# Autodesk Inventor assembly: ASSY,INTAKE,LINEAR
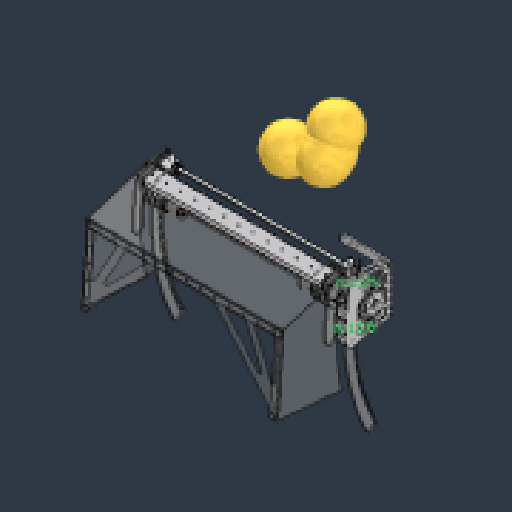
[picture p0: Inventor's stored thumbnail of the model, 512x512]
Saved by Autodesk Inventor 2026 (Build 300175050, 175E)
## iProperties
Created: 2026-04-11
Part Number: ASSY,INTAKE,LINEAR
Document SubType Name: Assembly
Designer: Jthib
Mass: 12352.9 g
Surface Area: 19154.1 cm^2
Volume: 9875.56 cm^3
Density: 1.25086 g/cm^3
Author: Jthib
## Documents named in this file (27)
- C:\Users\Jthib\Documents\GitHub\2026-Robot-Mechanical\LINEAR_INTAKE\ASSY,INTAKE,LINEAR.iam
- C:\Users\Jthib\Documents\GitHub\2026-Robot-Mechanical\#2_2026 Field CAD\GE-26900_ Fuel.ipt
- C:\Users\Jthib\Documents\GitHub\2026-Robot-Mechanical\Intake\PLATE,CLAMP,MK4i,Swerve,CUSTOM,FRC2026.ipt
- C:\Users\Jthib\Documents\GitHub\2026-Robot-Mechanical\LINEAR_INTAKE\PLATE,SIDE,INTAKE,FRONT.ipt
- C:\Users\Jthib\Documents\GitHub\2026-Robot-Mechanical\LINEAR_INTAKE\#old-linear-intake\INSIDE_INTAKE_PLATE.ipt
- C:\Users\Jthib\Documents\GitHub\2026-Robot-Mechanical\LINEAR_INTAKE\#old-linear-intake\FRONT_INTAKE_LEXAN.ipt
- C:\Users\Jthib\Documents\GitHub\2026-Robot-Mechanical\LINEAR_INTAKE\#old-linear-intake\SIDE_INTAKE_LEXAN.ipt
- C:\Users\Jthib\Documents\GitHub\2026-Robot-Mechanical\LINEAR_INTAKE\#old-linear-intake\SIDE_INTAKE_LEXAN_MIR.ipt
- C:\Users\Jthib\Documents\GitHub\2026-Robot-Mechanical\LINEAR_INTAKE\#old-linear-intake\TOP_INTAKE_LEXAN.ipt
- C:\Users\Jthib\Documents\GitHub\2026-Robot-Mechanical\#1_CAD Library\Power Transmission\Bearings\PURCHASED,HEX_BEARING.ipt
- C:\Users\Jthib\Documents\GitHub\2026-Robot-Mechanical\LINEAR_INTAKE\#old-linear-intake\INTAKE_DRIVEN_PULLY.ipt
- C:\Users\Jthib\Documents\GitHub\2026-Robot-Mechanical\LINEAR_INTAKE\#old-linear-intake\INSIDE_INTAKE_PLATE_MOTOR_MOUNT.ipt
- C:\Users\Jthib\Documents\GitHub\2026-Robot-Mechanical\LINEAR_INTAKE\#old-linear-intake\INSIDE_INTAKE_PLATE_MOTOR_MOUNT_MIR.ipt
- C:\Users\Jthib\Documents\GitHub\2026-Robot-Mechanical\LINEAR_INTAKE\#old-linear-intake\53t_Belt.ipt
- C:\Users\Jthib\Documents\GitHub\2026-Robot-Mechanical\LINEAR_INTAKE\#old-linear-intake\MOTOR_PLATE_PRINTED_SPACER.ipt
- C:\Users\Jthib\Documents\GitHub\2026-Robot-Mechanical\LINEAR_INTAKE\#old-linear-intake\OUTSIDE_INTAKE_SPACERS.ipt
- C:\Users\Jthib\Documents\GitHub\2026-Robot-Mechanical\LINEAR_INTAKE\#old-linear-intake\CRASH_BAR_INTAKE.ipt
- C:\Users\Jthib\Documents\GitHub\2026-Robot-Mechanical\#1_CAD Library\Electronics\CONTROLS,SPARK_FLEX.ipt
- C:\Users\Jthib\Documents\GitHub\2026-Robot-Mechanical\#1_CAD Library\Motors\MOTOR,REV,NEO,VORTEX.ipt
- C:\Users\Jthib\Documents\GitHub\2026-Robot-Mechanical\LINEAR_INTAKE\#old-linear-intake\INTAKE_DRIVER_PULLY.ipt
- C:\Users\Jthib\Documents\GitHub\2026-Robot-Mechanical\LINEAR_INTAKE\GEAR,PINION,INTAKE.ipt
- C:\Users\Jthib\Documents\GitHub\2026-Robot-Mechanical\Intake\STOCK,HEX,INTAKE.ipt
- C:\Users\Jthib\Documents\GitHub\2026-Robot-Mechanical\LINEAR_INTAKE\GEAR,DRIVE,INTAKE.ipt
- C:\Users\Jthib\Documents\GitHub\2026-Robot-Mechanical\LINEAR_INTAKE\SPACER,INTAKE,LINEAR.ipt
- C:\Users\Jthib\Documents\GitHub\2026-Robot-Mechanical\LINEAR_INTAKE\RACK,OUTSIDE.ipt
- C:\Users\Jthib\Documents\GitHub\2026-Robot-Mechanical\LINEAR_INTAKE\RACK,INSIDE.ipt
- C:\Users\Jthib\Documents\GitHub\2026-Robot-Mechanical\LINEAR_INTAKE\FRONT,HEX,INTAKE.ipt
## Components (42 placed, 26 different names)
1. PLATE,CLAMP,MK4i,Swerve,CUSTOM,FRC2026:1 — Mate:1, Mate:2, Mate:3, Mate:4, Mate:5
2. GE-26900_ Fuel:8
3. PLATE,SIDE,INTAKE,FRONT:1 — Mate:1, Mate:2, Mate:3, Flush:1, Mate:78, Mate:80, Mate:81, Mate:82, Mate:87, Mate:88, Mate:93
4. PLATE,SIDE,INTAKE,FRONT:2 — Mate:4, Flush:1, Mate:5, Mate:76, Insert:15
5. RACK,OUTSIDE:1 — Mate:76, Rotation:1, Rotation:2, Mate:89, Mate:90, Mate:91, Mate:93, Mate:99, Mate:100, Mate:101
6. INSIDE_INTAKE_PLATE:1 — Mate:38, Mate:41, Mate:42, Mate:49, Flush:21
7. INSIDE_INTAKE_PLATE:2 — Mate:31, Mate:47, Mate:49, Mate:79, Mate:92, Mate:105
8. FRONT_INTAKE_LEXAN:1 — Mate:73, Insert:7, Insert:8, Insert:9, Insert:10, Mate:97, Mate:98
9. SIDE_INTAKE_LEXAN:1 — Flush:20, Mate:97
10. SIDE_INTAKE_LEXAN_MIR:1 — Mate:98
11. TOP_INTAKE_LEXAN:1
12. PURCHASED,HEX_BEARING:1 — Mate:48, Mate:50, Mate:51
13. PURCHASED,HEX_BEARING:2 — Mate:48
14. INTAKE_DRIVEN_PULLY:1 — Mate:45
15. INSIDE_INTAKE_PLATE_MOTOR_MOUNT:1 — Mate:32, Mate:33, Mate:34, Mate:59, Mate:60, Mate:61, Insert:5, Insert:6
16. INSIDE_INTAKE_PLATE_MOTOR_MOUNT_MIR:1 — Mate:43, Mate:44, Insert:1, Insert:2, Mate:67, Insert:3, Insert:4
17. 53t_Belt:1 — Mate:45, Mate:68, Mate:69
18. 53t_Belt:2 — Mate:52, Mate:53, Mate:70, Mate:71
19. MOTOR_PLATE_PRINTED_SPACER:1 — Mate:38, Mate:41, Mate:42, Mate:43, Mate:44
20. MOTOR_PLATE_PRINTED_SPACER:2 — Mate:32, Mate:33, Mate:34, Mate:47
21. SPACER,INTAKE,LINEAR:1 — Mate:31, Mate:62, Mate:92, Mate:100, Mate:101, Mate:102
22. OUTSIDE_INTAKE_SPACERS:2
23. INTAKE_DRIVEN_PULLY:2 — Mate:50, Mate:51, Mate:52, Mate:53
24. CRASH_BAR_INTAKE:1 — Insert:3, Insert:4, Insert:5, Insert:6, Mate:73, Insert:7, Insert:8, Insert:9, Insert:10
25. CONTROLS,SPARK_FLEX:1 — Mate:59, Mate:60, Mate:61
26. MOTOR,REV,NEO,VORTEX:1
27. INTAKE_DRIVER_PULLY:1 — Mate:62, Mate:70, Mate:71
28. CONTROLS,SPARK_FLEX:2 — Insert:1, Insert:2
29. MOTOR,REV,NEO,VORTEX:2
30. INTAKE_DRIVER_PULLY:2 — Mate:67, Mate:68, Mate:69
31. PINION:1 — Mate:78, Rotation:1, Mate:82
32. STOCK,HEX,INTAKE:1 — Mate:79, Flush:20
33. PINION:2 — Mate:80, Mate:81, Rotation:2, Rotation:3
34. PURCHASED,HEX_BEARING:3 — Insert:15
35. GEAR,DRIVE,INTAKE:1 — Mate:87, Mate:88, Rotation:3
36. RACK,INSIDE:1 — Mate:89, Mate:90, Mate:91, Mate:99, Mate:102, Mate:103, Mate:104
37. RACK,OUTSIDE:2 — Mate:94, Mate:95, Mate:96
38. RACK,INSIDE:2 — Mate:94, Mate:95, Mate:96, Mate:103, Mate:104
39. GE-26900_ Fuel:9
40. GE-26900_ Fuel:10
41. GE-26900_ Fuel:11
42. FRONT,HEX,INTAKE:1 — Mate:105, Flush:21
## Relationships (103: Mate 76, Flush 13, Insert 11, RelateRotation 3)
- Mate:1: PLATE,CLAMP,MK4i,Swerve,CUSTOM,FRC2026:1 ↔ PLATE,SIDE,INTAKE,FRONT:1
- Mate:2 (0.127 mm): PLATE,CLAMP,MK4i,Swerve,CUSTOM,FRC2026:1 ↔ PLATE,SIDE,INTAKE,FRONT:1
- Mate:3 (0.1778 mm): PLATE,CLAMP,MK4i,Swerve,CUSTOM,FRC2026:1 ↔ PLATE,SIDE,INTAKE,FRONT:1
- Mate:4 (0.127 mm): PLATE,CLAMP,MK4i,Swerve,CUSTOM,FRC2026:1 ↔ PLATE,SIDE,INTAKE,FRONT:2
- Flush:1: PLATE,SIDE,INTAKE,FRONT:1 ↔ PLATE,SIDE,INTAKE,FRONT:2
- Mate:5: PLATE,CLAMP,MK4i,Swerve,CUSTOM,FRC2026:1 ↔ PLATE,SIDE,INTAKE,FRONT:2
- [Mate]: FRONT_INTAKE_LEXAN:1 ↔ SIDE_INTAKE_LEXAN:1
- [Flush]: FRONT_INTAKE_LEXAN:1 ↔ SIDE_INTAKE_LEXAN:1
- [Mate]: FRONT_INTAKE_LEXAN:1 ↔ SIDE_INTAKE_LEXAN_MIR:1
- [Flush]: FRONT_INTAKE_LEXAN:1 ↔ SIDE_INTAKE_LEXAN_MIR:1
- [Mate]: SIDE_INTAKE_LEXAN_MIR:1 ↔ TOP_INTAKE_LEXAN:1
- [Flush]: SIDE_INTAKE_LEXAN_MIR:1 ↔ TOP_INTAKE_LEXAN:1
- [Flush]: FRONT_INTAKE_LEXAN:1 ↔ TOP_INTAKE_LEXAN:1
- [Mate]: INSIDE_INTAKE_PLATE:2 ↔ PURCHASED,HEX_BEARING:1
- [Mate]: INSIDE_INTAKE_PLATE:2 ↔ PURCHASED,HEX_BEARING:1
- [Mate]: INSIDE_INTAKE_PLATE:1 ↔ PURCHASED,HEX_BEARING:2
- [Mate]: INSIDE_INTAKE_PLATE:1 ↔ PURCHASED,HEX_BEARING:2
- [Mate] (0.7937 mm): PURCHASED,HEX_BEARING:2 ↔ INTAKE_DRIVEN_PULLY:1
- [Mate]: PURCHASED,HEX_BEARING:2 ↔ INTAKE_DRIVEN_PULLY:1
- [Mate]: INTAKE_DRIVEN_PULLY:1 ↔ 53t_Belt:1
- [Mate]: INSIDE_INTAKE_PLATE_MOTOR_MOUNT_MIR:1 ↔ MOTOR_PLATE_PRINTED_SPACER:1
- [Mate]: INSIDE_INTAKE_PLATE:2 ↔ MOTOR_PLATE_PRINTED_SPACER:2
- [Flush]: INSIDE_INTAKE_PLATE:2 ↔ MOTOR_PLATE_PRINTED_SPACER:2
- [Flush]: INSIDE_INTAKE_PLATE_MOTOR_MOUNT_MIR:1 ↔ MOTOR_PLATE_PRINTED_SPACER:1
- [Flush]: INSIDE_INTAKE_PLATE:2 ↔ SPACER,INTAKE,LINEAR:1
- [Flush]: MOTOR_PLATE_PRINTED_SPACER:2 ↔ SPACER,INTAKE,LINEAR:1
- [Mate]: INSIDE_INTAKE_PLATE:1 ↔ OUTSIDE_INTAKE_SPACERS:2
- [Flush]: INSIDE_INTAKE_PLATE:1 ↔ OUTSIDE_INTAKE_SPACERS:2
- [Flush]: MOTOR_PLATE_PRINTED_SPACER:1 ↔ OUTSIDE_INTAKE_SPACERS:2
- Mate:31: INSIDE_INTAKE_PLATE:2 ↔ SPACER,INTAKE,LINEAR:1
- Mate:32: INSIDE_INTAKE_PLATE_MOTOR_MOUNT:1 ↔ MOTOR_PLATE_PRINTED_SPACER:2
- Mate:33: INSIDE_INTAKE_PLATE_MOTOR_MOUNT:1 ↔ MOTOR_PLATE_PRINTED_SPACER:2
- Mate:34: INSIDE_INTAKE_PLATE_MOTOR_MOUNT:1 ↔ MOTOR_PLATE_PRINTED_SPACER:2
- Mate:38: INSIDE_INTAKE_PLATE:1 ↔ MOTOR_PLATE_PRINTED_SPACER:1
- Mate:41: INSIDE_INTAKE_PLATE:1 ↔ MOTOR_PLATE_PRINTED_SPACER:1
- Mate:42: INSIDE_INTAKE_PLATE:1 ↔ MOTOR_PLATE_PRINTED_SPACER:1
- Mate:43: INSIDE_INTAKE_PLATE_MOTOR_MOUNT_MIR:1 ↔ MOTOR_PLATE_PRINTED_SPACER:1
- Mate:44: INSIDE_INTAKE_PLATE_MOTOR_MOUNT_MIR:1 ↔ MOTOR_PLATE_PRINTED_SPACER:1
- Mate:45: INTAKE_DRIVEN_PULLY:1 ↔ 53t_Belt:1
- Mate:47: INSIDE_INTAKE_PLATE:2 ↔ MOTOR_PLATE_PRINTED_SPACER:2
- Mate:48: PURCHASED,HEX_BEARING:1 ↔ PURCHASED,HEX_BEARING:2
- Mate:49: INSIDE_INTAKE_PLATE:1 ↔ INSIDE_INTAKE_PLATE:2
- Mate:50: PURCHASED,HEX_BEARING:1 ↔ INTAKE_DRIVEN_PULLY:2
- Mate:51: PURCHASED,HEX_BEARING:1 ↔ INTAKE_DRIVEN_PULLY:2
- Mate:52: 53t_Belt:2 ↔ INTAKE_DRIVEN_PULLY:2
- Mate:53: 53t_Belt:2 ↔ INTAKE_DRIVEN_PULLY:2
- [Mate]: CONTROLS,SPARK_FLEX:1 ↔ MOTOR,REV,NEO,VORTEX:1
- [Mate]: CONTROLS,SPARK_FLEX:1 ↔ MOTOR,REV,NEO,VORTEX:1
- [Mate]: CONTROLS,SPARK_FLEX:1 ↔ MOTOR,REV,NEO,VORTEX:1
- Mate:59: INSIDE_INTAKE_PLATE_MOTOR_MOUNT:1 ↔ CONTROLS,SPARK_FLEX:1
- Mate:60: INSIDE_INTAKE_PLATE_MOTOR_MOUNT:1 ↔ CONTROLS,SPARK_FLEX:1
- Mate:61: INSIDE_INTAKE_PLATE_MOTOR_MOUNT:1 ↔ CONTROLS,SPARK_FLEX:1
- Mate:62: SPACER,INTAKE,LINEAR:1 ↔ INTAKE_DRIVER_PULLY:1
- [Mate]: CONTROLS,SPARK_FLEX:2 ↔ MOTOR,REV,NEO,VORTEX:2
- [Mate]: CONTROLS,SPARK_FLEX:2 ↔ MOTOR,REV,NEO,VORTEX:2
- [Mate]: CONTROLS,SPARK_FLEX:2 ↔ MOTOR,REV,NEO,VORTEX:2
- Insert:1: INSIDE_INTAKE_PLATE_MOTOR_MOUNT_MIR:1 ↔ CONTROLS,SPARK_FLEX:2
- Insert:2: INSIDE_INTAKE_PLATE_MOTOR_MOUNT_MIR:1 ↔ CONTROLS,SPARK_FLEX:2
- Mate:67: INSIDE_INTAKE_PLATE_MOTOR_MOUNT_MIR:1 ↔ INTAKE_DRIVER_PULLY:2
- Mate:68: 53t_Belt:1 ↔ INTAKE_DRIVER_PULLY:2
- Mate:69: 53t_Belt:1 ↔ INTAKE_DRIVER_PULLY:2
- Mate:70: 53t_Belt:2 ↔ INTAKE_DRIVER_PULLY:1
- Mate:71: 53t_Belt:2 ↔ INTAKE_DRIVER_PULLY:1
- Insert:3: INSIDE_INTAKE_PLATE_MOTOR_MOUNT_MIR:1 ↔ CRASH_BAR_INTAKE:1
- Insert:4: INSIDE_INTAKE_PLATE_MOTOR_MOUNT_MIR:1 ↔ CRASH_BAR_INTAKE:1
- Insert:5: INSIDE_INTAKE_PLATE_MOTOR_MOUNT:1 ↔ CRASH_BAR_INTAKE:1
- Insert:6: INSIDE_INTAKE_PLATE_MOTOR_MOUNT:1 ↔ CRASH_BAR_INTAKE:1
- Mate:73: FRONT_INTAKE_LEXAN:1 ↔ CRASH_BAR_INTAKE:1
- Insert:7: FRONT_INTAKE_LEXAN:1 ↔ CRASH_BAR_INTAKE:1
- Insert:8: FRONT_INTAKE_LEXAN:1 ↔ CRASH_BAR_INTAKE:1
- Insert:9: FRONT_INTAKE_LEXAN:1 ↔ CRASH_BAR_INTAKE:1
- Insert:10: FRONT_INTAKE_LEXAN:1 ↔ CRASH_BAR_INTAKE:1
- Mate:76: PLATE,SIDE,INTAKE,FRONT:2 ↔ RACK,OUTSIDE:1
- Mate:78: PLATE,SIDE,INTAKE,FRONT:1 ↔ PINION:1
- Rotation:1 [RelateRotation] (0.0261 ul): RACK,OUTSIDE:1 ↔ PINION:1
- Mate:79: INSIDE_INTAKE_PLATE:2 ↔ STOCK,HEX,INTAKE:1
- Flush:20: SIDE_INTAKE_LEXAN:1 ↔ STOCK,HEX,INTAKE:1
- Mate:80: PLATE,SIDE,INTAKE,FRONT:1 ↔ PINION:2
- Mate:81: PLATE,SIDE,INTAKE,FRONT:1 ↔ PINION:2
- Rotation:2 [RelateRotation] (0.0261 ul): RACK,OUTSIDE:1 ↔ PINION:2
- Mate:82: PLATE,SIDE,INTAKE,FRONT:1 ↔ PINION:1
- Insert:15: PLATE,SIDE,INTAKE,FRONT:2 ↔ PURCHASED,HEX_BEARING:3
- Mate:87: PLATE,SIDE,INTAKE,FRONT:1 ↔ GEAR,DRIVE,INTAKE:1
- Mate:88: PLATE,SIDE,INTAKE,FRONT:1 ↔ GEAR,DRIVE,INTAKE:1
- Rotation:3 [RelateRotation] (2 ul): PINION:2 ↔ GEAR,DRIVE,INTAKE:1
- Mate:89: RACK,OUTSIDE:1 ↔ RACK,INSIDE:1
- Mate:90: RACK,OUTSIDE:1 ↔ RACK,INSIDE:1
- Mate:91: RACK,OUTSIDE:1 ↔ RACK,INSIDE:1
- Mate:92: INSIDE_INTAKE_PLATE:2 ↔ SPACER,INTAKE,LINEAR:1
- Mate:93: PLATE,SIDE,INTAKE,FRONT:1 ↔ RACK,OUTSIDE:1
- Mate:94: RACK,OUTSIDE:2 ↔ RACK,INSIDE:2
- Mate:95: RACK,OUTSIDE:2 ↔ RACK,INSIDE:2
- Mate:96: RACK,OUTSIDE:2 ↔ RACK,INSIDE:2
- Mate:97: FRONT_INTAKE_LEXAN:1 ↔ SIDE_INTAKE_LEXAN:1
- Mate:98: FRONT_INTAKE_LEXAN:1 ↔ SIDE_INTAKE_LEXAN_MIR:1
- Mate:99: RACK,OUTSIDE:1 ↔ RACK,INSIDE:1
- Mate:100: RACK,OUTSIDE:1 ↔ SPACER,INTAKE,LINEAR:1
- Mate:101: RACK,OUTSIDE:1 ↔ SPACER,INTAKE,LINEAR:1
- Mate:102: SPACER,INTAKE,LINEAR:1 ↔ RACK,INSIDE:1
- Mate:103: RACK,INSIDE:1 ↔ RACK,INSIDE:2
- Mate:104: RACK,INSIDE:1 ↔ RACK,INSIDE:2
- Mate:105: INSIDE_INTAKE_PLATE:2 ↔ FRONT,HEX,INTAKE:1
- Flush:21: INSIDE_INTAKE_PLATE:1 ↔ FRONT,HEX,INTAKE:1
## Named parameters: d544_d534_d406_d72_d163_d8 = 0 mm, d545_d535_d407_d73_d164_d9 = 0 mm, d546_d536_d408_d74_d165_d10 = 0 mm, d87_d544_d534_d406_d72_d163_d8 = 0 mm, d88_d545_d535_d407_d73_d164_d9 = 0 mm, d89_d546_d536_d408_d74_d165_d10 = 0 mm
